# Autodesk Inventor assembly: SansRotor_Ricea f. Florentina alexandra-T7
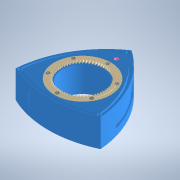
[picture p0: Inventor's stored thumbnail of the model, 180x180]
Saved by Autodesk Inventor 2022 (Build 260153000, 153)
## iProperties
Student_ACE: Ricea f. Florentina alexandra
Grupa_ACE: CR-3
Tema_ACE: 7-Ansamblu motor Wankel
An_ACE: 2022
Created: 2022-02-18
Part Number: SansRotor_Ricea f. Florentina alexandra-T7
Document SubType Name: Assembly
Designer: mtrot
Author: mtrot
## Documents named in this file (4)
- C:\1.GAC\tema7_var2\SansRotor_Ricea f. Florentina alexandra-T7.iam
- C:\1.GAC\tema7_var2\Rotor.ipt
- C:\1.GAC\tema7_var2\Roata.ipt
- C:\1.GAC\tema7_var2\SubAns-M4.iam
## Components (3 placed, 3 different names)
1. Rotor:1 — Mate:1, Mate:2, Mate:3, Mate:4, Mate:5, Angle:1
2. Roata:1 — Mate:4, Mate:5, Angle:1
3. SubAns-M4:1 [sub-assembly]
## Relationships (7: Mate 5, Angle 1, Insert 1)
- Mate:1: Rotor:1
- Mate:2: Rotor:1
- Mate:3: Rotor:1
- Mate:4: Rotor:1 ↔ Roata:1
- Mate:5: Rotor:1 ↔ Roata:1
- Angle:1 (0 deg): Rotor:1 ↔ Roata:1
- [Insert]: Roata:1 ↔ SubAns-M4:1
